# Autodesk Inventor assembly: Slidey Mecanum L thing V2
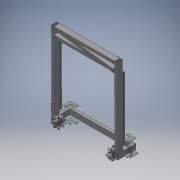
[picture p0: Inventor's stored thumbnail of the model, 180x180]
Saved by Autodesk Inventor 2018 (Build 220112000, 112)
## iProperties
Created: 2019-01-11
Part Number: Slidey Mecanum L thing V2
Document SubType Name: Assembly
Designer: s-2512711
Author: s-2512711
## Documents named in this file (11)
- \\studenthome\students\S-2512711\GitHub\2019CAD\Drivebase but Calvin is a mad man\Slidey Mecanum L thing V2.iam
- \\studenthome\students\S-2512711\GitHub\2019CAD\Drivebase but Calvin is a mad man\1X2 7in.ipt
- \\studenthome\students\S-2512711\GitHub\2019CAD\Drivebase but Calvin is a mad man\1x2 28in.ipt
- \\studenthome\students\S-2512711\GitHub\2019CAD\Drivebase but Calvin is a mad man\1x2 30in.ipt
- \\studenthome\students\S-2512711\GitHub\2019CAD\Drivebase but Calvin is a mad man\4_Mecanum_Wheel_Left_217-3644.iam
- \\studenthome\students\S-2512711\GitHub\2019CAD\Drivebase but Calvin is a mad man\4_Mecanum_Wheel_Right_217-3645.iam
- \\studenthome\students\S-2512711\GitHub\2019CAD\Drivebase but Calvin is a mad man\Strutural Integrity Bar.ipt
- \\studenthome\students\S-2512711\GitHub\2019CAD\Drivebase but Calvin is a mad man\WS_10_40_610_4.ipt
- \\studenthome\students\S-2512711\GitHub\2019CAD\Drivebase but Calvin is a mad man\91831A011_TYPE 18-8 STAINLESS STL NYLON-INSERT LOCKNUT.ipt
- \\studenthome\students\S-2512711\GitHub\2019CAD\Drivebase but Calvin is a mad man\73434-Fastenal-01-12-2019.ipt
- \\studenthome\students\S-2512711\GitHub\2019CAD\Drivebase but Calvin is a mad man\L gusset.ipt
## Components (37 placed, 10 different names)
1. 1X2 7in:1 — Mate:4, Mate:5, Mate:6, Mate:7, Mate:8, Mate:9, Mate:22, Mate:23, Mate:24
2. 1X2 7in:2 — Mate:1, Mate:2, Mate:3, Mate:10, Mate:11, Mate:12, Mate:25, Mate:26, Mate:27
3. 1x2 28in:1 — Mate:7, Mate:8, Mate:9, Mate:10, Mate:11, Mate:12
4. 1x2 28in:2 — Mate:16, Mate:17, Flush:1, Mate:29, Mate:31, Mate:39, Mate:44, Mate:46
5. 1x2 28in:3 — Mate:13, Mate:14, Mate:15, Flush:1, Mate:18, Mate:19, Mate:20, Mate:21, Mate:35, Rotation:2, Mate:48
6. 1x2 30in:1 — Mate:4, Mate:5, Mate:6, Mate:28, Flush:2
7. 1x2 30in:2 — Mate:1, Mate:2, Mate:3, Mate:13, Mate:14, Mate:15, Mate:16, Mate:17, Mate:30, Flush:3
8. 4_Mecanum_Wheel_Left_217-3644:1 [sub-assembly] — Mate:22, Mate:23, Mate:24
9. 4_Mecanum_Wheel_Right_217-3645:1 [sub-assembly] — Mate:25, Mate:26, Mate:27
10. Strutural Integrity Bar:1 — Mate:18, Mate:19, Mate:40, Mate:41, Mate:43
11. Strutural Integrity Bar:2 — Mate:20, Mate:21, Mate:32, Mate:33, Rotation:3, Mate:36, Mate:37
12. WS_10_40_610_4:1 — Mate:30, Mate:31, Flush:3
13. WS_10_40_610_4:2 — Mate:28, Mate:29, Flush:2
14. 91831A011_TYPE 18-8 STAINLESS STL NYLON-INSERT LOCKNUT:1 — Mate:34, Mate:35, Rotation:2
15. 91831A011_TYPE 18-8 STAINLESS STL NYLON-INSERT LOCKNUT:2 — Mate:38, Mate:39
16. 73434-Fastenal-01-12-2019:1 — Mate:36, Mate:37, Mate:38
17. 73434-Fastenal-01-12-2019:2 — Mate:32, Mate:33, Mate:34, Rotation:3
18. 73434-Fastenal-01-12-2019:3 — Mate:43, Mate:44, Mate:45
19. 73434-Fastenal-01-12-2019:4 — Mate:40, Mate:41, Mate:47
20. 91831A011_TYPE 18-8 STAINLESS STL NYLON-INSERT LOCKNUT:3 — Mate:47, Mate:48
21. 91831A011_TYPE 18-8 STAINLESS STL NYLON-INSERT LOCKNUT:4 — Mate:45, Mate:46
22. 91831A011_TYPE 18-8 STAINLESS STL NYLON-INSERT LOCKNUT:5
23. 91831A011_TYPE 18-8 STAINLESS STL NYLON-INSERT LOCKNUT:6
24. 91831A011_TYPE 18-8 STAINLESS STL NYLON-INSERT LOCKNUT:7
25. 91831A011_TYPE 18-8 STAINLESS STL NYLON-INSERT LOCKNUT:8
26. 91831A011_TYPE 18-8 STAINLESS STL NYLON-INSERT LOCKNUT:9
27. 91831A011_TYPE 18-8 STAINLESS STL NYLON-INSERT LOCKNUT:10
28. 73434-Fastenal-01-12-2019:5
29. 73434-Fastenal-01-12-2019:6
30. 73434-Fastenal-01-12-2019:7
31. 73434-Fastenal-01-12-2019:8
32. 73434-Fastenal-01-12-2019:9
33. 73434-Fastenal-01-12-2019:10
34. L gusset:1
35. L gusset:2
36. L gusset:3
37. L gusset:4
## Relationships (52: Mate 47, Flush 3, RelateRotation 2)
- Mate:1: 1X2 7in:2 ↔ 1x2 30in:2
- Mate:2: 1X2 7in:2 ↔ 1x2 30in:2
- Mate:3: 1X2 7in:2 ↔ 1x2 30in:2
- Mate:4: 1X2 7in:1 ↔ 1x2 30in:1
- Mate:5: 1X2 7in:1 ↔ 1x2 30in:1
- Mate:6: 1X2 7in:1 ↔ 1x2 30in:1
- Mate:7: 1X2 7in:1 ↔ 1x2 28in:1
- Mate:8: 1X2 7in:1 ↔ 1x2 28in:1
- Mate:9: 1X2 7in:1 ↔ 1x2 28in:1
- Mate:10: 1X2 7in:2 ↔ 1x2 28in:1
- Mate:11: 1X2 7in:2 ↔ 1x2 28in:1
- Mate:12: 1X2 7in:2 ↔ 1x2 28in:1
- Mate:13: 1x2 28in:3 ↔ 1x2 30in:2
- Mate:14: 1x2 28in:3 ↔ 1x2 30in:2
- Mate:15: 1x2 28in:3 ↔ 1x2 30in:2
- Mate:16: 1x2 28in:2 ↔ 1x2 30in:2
- Mate:17: 1x2 28in:2 ↔ 1x2 30in:2
- Flush:1 (69.85 mm): 1x2 28in:2 ↔ 1x2 28in:3
- Mate:18: 1x2 28in:3 ↔ Strutural Integrity Bar:1
- Mate:19: 1x2 28in:3 ↔ Strutural Integrity Bar:1
- Mate:20: 1x2 28in:3 ↔ Strutural Integrity Bar:2
- Mate:21: 1x2 28in:3 ↔ Strutural Integrity Bar:2
- Mate:22: 1X2 7in:1 ↔ 4_Mecanum_Wheel_Left_217-3644:1
- Mate:23: 1X2 7in:1 ↔ 4_Mecanum_Wheel_Left_217-3644:1
- Mate:24: 1X2 7in:1 ↔ 4_Mecanum_Wheel_Left_217-3644:1
- Mate:25: 1X2 7in:2 ↔ 4_Mecanum_Wheel_Right_217-3645:1
- Mate:26: 1X2 7in:2 ↔ 4_Mecanum_Wheel_Right_217-3645:1
- Mate:27: 1X2 7in:2 ↔ 4_Mecanum_Wheel_Right_217-3645:1
- Mate:28: 1x2 30in:1 ↔ WS_10_40_610_4:2
- Mate:29 (6.35 mm): 1x2 28in:2 ↔ WS_10_40_610_4:2
- Flush:2 (-7.3025 mm): 1x2 30in:1 ↔ WS_10_40_610_4:2
- Mate:30: 1x2 30in:2 ↔ WS_10_40_610_4:1
- Mate:31 (6.35 mm): 1x2 28in:2 ↔ WS_10_40_610_4:1
- Flush:3 (-7.3025 mm): 1x2 30in:2 ↔ WS_10_40_610_4:1
- Mate:32: Strutural Integrity Bar:2 ↔ 73434-Fastenal-01-12-2019:2
- Mate:33: Strutural Integrity Bar:2 ↔ 73434-Fastenal-01-12-2019:2
- Mate:34: 91831A011_TYPE 18-8 STAINLESS STL NYLON-INSERT LOCKNUT:1 ↔ 73434-Fastenal-01-12-2019:2
- Mate:35: 1x2 28in:3 ↔ 91831A011_TYPE 18-8 STAINLESS STL NYLON-INSERT LOCKNUT:1
- Rotation:2 [RelateRotation] (1 ul): 1x2 28in:3 ↔ 91831A011_TYPE 18-8 STAINLESS STL NYLON-INSERT LOCKNUT:1
- Rotation:3 [RelateRotation] (1 ul): Strutural Integrity Bar:2 ↔ 73434-Fastenal-01-12-2019:2
- Mate:36: Strutural Integrity Bar:2 ↔ 73434-Fastenal-01-12-2019:1
- Mate:37: Strutural Integrity Bar:2 ↔ 73434-Fastenal-01-12-2019:1
- Mate:38: 91831A011_TYPE 18-8 STAINLESS STL NYLON-INSERT LOCKNUT:2 ↔ 73434-Fastenal-01-12-2019:1
- Mate:39: 1x2 28in:2 ↔ 91831A011_TYPE 18-8 STAINLESS STL NYLON-INSERT LOCKNUT:2
- Mate:40: Strutural Integrity Bar:1 ↔ 73434-Fastenal-01-12-2019:4
- Mate:41: Strutural Integrity Bar:1 ↔ 73434-Fastenal-01-12-2019:4
- Mate:43: Strutural Integrity Bar:1 ↔ 73434-Fastenal-01-12-2019:3
- Mate:44: 1x2 28in:2 ↔ 73434-Fastenal-01-12-2019:3
- Mate:45: 73434-Fastenal-01-12-2019:3 ↔ 91831A011_TYPE 18-8 STAINLESS STL NYLON-INSERT LOCKNUT:4
- Mate:46: 1x2 28in:2 ↔ 91831A011_TYPE 18-8 STAINLESS STL NYLON-INSERT LOCKNUT:4
- Mate:47: 73434-Fastenal-01-12-2019:4 ↔ 91831A011_TYPE 18-8 STAINLESS STL NYLON-INSERT LOCKNUT:3
- Mate:48: 1x2 28in:3 ↔ 91831A011_TYPE 18-8 STAINLESS STL NYLON-INSERT LOCKNUT:3
